# Autodesk Inventor assembly: New_battery
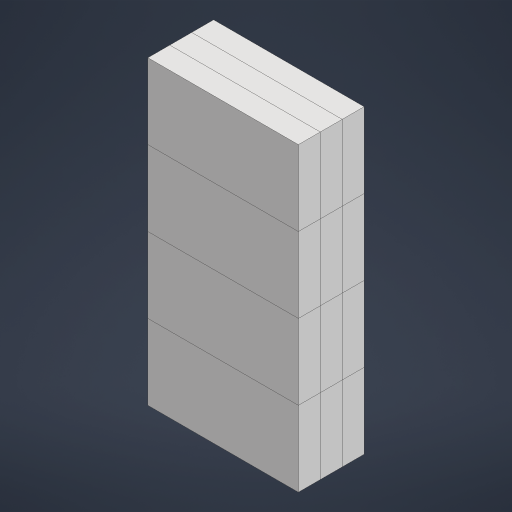
[picture p0: Inventor's stored thumbnail of the model, 512x512]
Saved by Autodesk Inventor 2024 (Build 280153000, 153)
## iProperties
Created: 2024-02-29
Part Number: New_battery
Document SubType Name: Assembly
Designer: calvi
Author: calvi
## Documents named in this file (2)
- C:\Users\calvi\OneDrive\Robocup Rescue\Chassis\Electronics Box\EBox-Parts\New_battery.iam
- C:\Users\calvi\OneDrive\Robocup Rescue\Chassis\Electronics Box\EBox-Parts\Battery_Cell.ipt
## Components (12 placed, 1 different names)
1. Battery_Cell:1 — Mate:8, Flush:15, Flush:17, Mate:10, Flush:19, Flush:20
2. Battery_Cell:2 — Mate:6, Mate:7, Flush:11, Flush:12, Flush:13, Flush:14
3. Battery_Cell:3 — Mate:7, Flush:12, Flush:13
4. Battery_Cell:4 — Mate:9, Flush:16, Flush:18
5. Battery_Cell:5 — Mate:8, Mate:9, Flush:15, Flush:16, Flush:17, Flush:18
6. Battery_Cell:6 — Mate:4, Flush:5, Flush:8
7. Battery_Cell:7 — Mate:3, Flush:6, Flush:7, Mate:5, Flush:9, Flush:10
8. Battery_Cell:8 — Mate:3, Mate:4, Flush:5, Flush:6, Flush:7, Flush:8
9. Battery_Cell:9 — Mate:1, Flush:1, Flush:4, Mate:5, Flush:9, Flush:10, Mate:11, Flush:21, Flush:22
10. Battery_Cell:10 — Mate:6, Flush:11, Flush:14, Mate:10, Flush:19, Flush:20, Mate:11, Flush:21, Flush:22
11. Battery_Cell:11 — Mate:2, Flush:2, Flush:3
12. Battery_Cell:12 — Mate:1, Mate:2, Flush:1, Flush:2, Flush:3, Flush:4
## Relationships (33: Flush 22, Mate 11)
- Mate:1: Battery_Cell:9 ↔ Battery_Cell:12
- Mate:2: Battery_Cell:11 ↔ Battery_Cell:12
- Flush:1: Battery_Cell:9 ↔ Battery_Cell:12
- Flush:2: Battery_Cell:11 ↔ Battery_Cell:12
- Flush:3: Battery_Cell:11 ↔ Battery_Cell:12
- Flush:4: Battery_Cell:9 ↔ Battery_Cell:12
- Mate:3: Battery_Cell:7 ↔ Battery_Cell:8
- Mate:4: Battery_Cell:6 ↔ Battery_Cell:8
- Flush:5: Battery_Cell:6 ↔ Battery_Cell:8
- Flush:6: Battery_Cell:7 ↔ Battery_Cell:8
- Flush:7: Battery_Cell:7 ↔ Battery_Cell:8
- Flush:8: Battery_Cell:6 ↔ Battery_Cell:8
- Mate:5: Battery_Cell:7 ↔ Battery_Cell:9
- Flush:9: Battery_Cell:7 ↔ Battery_Cell:9
- Flush:10: Battery_Cell:7 ↔ Battery_Cell:9
- Mate:6: Battery_Cell:2 ↔ Battery_Cell:10
- Mate:7: Battery_Cell:2 ↔ Battery_Cell:3
- Flush:11: Battery_Cell:2 ↔ Battery_Cell:10
- Flush:12: Battery_Cell:2 ↔ Battery_Cell:3
- Flush:13: Battery_Cell:2 ↔ Battery_Cell:3
- Flush:14: Battery_Cell:2 ↔ Battery_Cell:10
- Mate:8: Battery_Cell:1 ↔ Battery_Cell:5
- Mate:9: Battery_Cell:4 ↔ Battery_Cell:5
- Flush:15: Battery_Cell:1 ↔ Battery_Cell:5
- Flush:16: Battery_Cell:4 ↔ Battery_Cell:5
- Flush:17: Battery_Cell:1 ↔ Battery_Cell:5
- Flush:18: Battery_Cell:4 ↔ Battery_Cell:5
- Mate:10: Battery_Cell:1 ↔ Battery_Cell:10
- Flush:19: Battery_Cell:1 ↔ Battery_Cell:10
- Flush:20: Battery_Cell:1 ↔ Battery_Cell:10
- Mate:11: Battery_Cell:9 ↔ Battery_Cell:10
- Flush:21: Battery_Cell:9 ↔ Battery_Cell:10
- Flush:22: Battery_Cell:9 ↔ Battery_Cell:10
